# Autodesk Inventor assembly: First Design
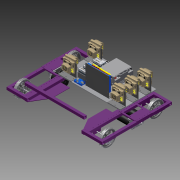
[picture p0: Inventor's stored thumbnail of the model, 180x180]
Saved by Autodesk Inventor 2012 (Build 160160000, 160)
## iProperties
Created: 2012-01-09
Part Number: First Design
Document SubType Name: Assembly
Designer: William
Author: William
## Documents named in this file (12)
- C:\Users\William\Dropbox\Robotics\CAD\team1885frc\Robot2012\Concepts\Electronics Board\First Design.iam
- C:\Users\William\Dropbox\Robotics\CAD\team1885frc\Robot2012\DriveTrain\DiveTrain_FullAssembly.iam
- C:\Users\William\Dropbox\Robotics\CAD\team1885frc\Robot2012\Concepts\Electronics Board\24in-by-14in_electronics_board.ipt
- C:\Users\William\Dropbox\Robotics\CAD\team1885frc\Electronics\Jag\Jag.iam
- C:\Users\William\Dropbox\Robotics\CAD\team1885frc\Electronics\DigitalSidecar\elc_Digital_Sidecar_inv.iam
- C:\Users\William\Dropbox\Robotics\CAD\team1885frc\Electronics\PowerDistributionBoard\elc_Power_Distro_inv.iam
- C:\Users\William\Dropbox\Robotics\CAD\team1885frc\Electronics\Battery.ipt
- C:\Users\William\Dropbox\Robotics\CAD\team1885frc\Robot2012\Concepts\Electronics Board\BatteryMountSide.ipt
- C:\Users\William\Dropbox\Robotics\CAD\team1885frc\Electronics\cRIO_7Slot\NI Controller.iam
- C:\Users\William\Dropbox\Robotics\CAD\team1885frc\Electronics\Breaker\Breaker.iam
- C:\Users\William\Dropbox\Robotics\CAD\team1885frc\Electronics\dualjaguarstand.ipt
- C:\Users\William\Dropbox\Robotics\CAD\team1885frc\Robot2012\Concepts\Electronics Board\PowerDistributionStandmount.ipt
## Components (27 placed, 11 different names)
1. DiveTrain_FullAssembly:1 [sub-assembly] — Flush:2, Angle:1, Angle:9, Flush:27
2. 24in-by-14in_electronics_board:1 — Flush:2, Mate:12, Mate:15, Mate:16, Flush:8, Flush:10, Flush:11, Mate:28, Flush:12, Mate:47, Flush:17, Flush:18, Mate:51, Flush:19, Mate:55, Flush:20, Flush:21, Mate:60, Flush:22, Flush:23, Mate:64, Flush:24, Flush:25, Mate:71, Flush:26, Flush:27
3. Jag:1 [sub-assembly] — Mate:26, Mate:42, Mate:54, Mate:56, Mate:58
4. Jag:2 [sub-assembly] — Mate:27, Mate:41, Mate:53
5. Jag:3 [sub-assembly] — Mate:31, Mate:40, Mate:49, Flush:18
6. Jag:4 [sub-assembly] — Mate:31, Mate:40, Mate:46, Mate:48, Angle:4
7. Jag:5 [sub-assembly] — Mate:35, Mate:39, Mate:65, Mate:66, Mate:67
8. Jag:6 [sub-assembly] — Mate:37, Mate:38, Mate:59, Mate:62, Angle:7
9. Jag:7 [sub-assembly] — Mate:37, Mate:38, Mate:61, Flush:23
10. Jag:8 [sub-assembly] — Mate:27, Mate:41, Mate:50, Mate:52, Mate:58, Angle:5
11. Jag:9 [sub-assembly] — Mate:26, Mate:42, Mate:57, Angle:6
12. Jag:10 [sub-assembly] — Mate:35, Mate:39, Mate:63, Angle:8
13. elc_Digital_Sidecar_inv:1 [sub-assembly] — Mate:15, Flush:10
14. elc_Power_Distro_inv:1 [sub-assembly] — Mate:68, Mate:69, Mate:70
15. Battery:1 — Mate:2, Mate:3, Mate:4, Mate:5, Mate:6, Mate:7, Mate:8, Mate:9, Mate:10, Mate:11, Flush:3, Flush:4
16. BatteryMountSide:1 — Mate:3, Mate:4, Mate:10
17. BatteryMountSide:2 — Mate:6, Mate:9, Mate:11
18. BatteryMountSide:3 — Mate:2, Mate:5, Flush:3
19. BatteryMountSide:4 — Mate:7, Mate:8, Flush:4, Mate:12, Angle:1, Flush:11
20. NI Controller:1 [sub-assembly] — Mate:16, Flush:8
21. Breaker:1 [sub-assembly] — Mate:28, Flush:12
22. dualjaguarstand:1 — Mate:46, Mate:47, Flush:17, Mate:48, Mate:49, Angle:4
23. dualjaguarstand:2 — Mate:50, Mate:51, Mate:52, Mate:53, Flush:19, Angle:5
24. dualjaguarstand:3 — Mate:54, Mate:55, Mate:56, Mate:57, Flush:20, Flush:21, Angle:6
25. dualjaguarstand:4 — Mate:63, Mate:64, Mate:65, Mate:66, Mate:67, Flush:24, Flush:25, Angle:8
26. dualjaguarstand:5 — Mate:59, Mate:60, Flush:22, Mate:61, Mate:62, Angle:7
27. PowerDistributionStandmount:1 — Mate:68, Mate:69, Mate:70, Mate:71, Angle:9, Flush:26
## Relationships (75: Mate 50, Flush 18, Angle 7)
- Flush:2 (-12.7 mm): DiveTrain_FullAssembly:1 ↔ 24in-by-14in_electronics_board:1
- Mate:2 (5.08 mm): Battery:1 ↔ BatteryMountSide:3
- Mate:3 (5.08 mm): Battery:1 ↔ BatteryMountSide:1
- Mate:4: Battery:1 ↔ BatteryMountSide:1
- Mate:5: Battery:1 ↔ BatteryMountSide:3
- Mate:6: Battery:1 ↔ BatteryMountSide:2
- Mate:7: Battery:1 ↔ BatteryMountSide:4
- Mate:8 (5.08 mm): Battery:1 ↔ BatteryMountSide:4
- Mate:9: Battery:1 ↔ BatteryMountSide:2
- Mate:10 (16.51 mm): Battery:1 ↔ BatteryMountSide:1
- Mate:11 (16.51 mm): Battery:1 ↔ BatteryMountSide:2
- Flush:3 (-12.446 mm): Battery:1 ↔ BatteryMountSide:3
- Flush:4 (12.446 mm): Battery:1 ↔ BatteryMountSide:4
- Mate:12: 24in-by-14in_electronics_board:1 ↔ BatteryMountSide:4
- Mate:15: 24in-by-14in_electronics_board:1 ↔ elc_Digital_Sidecar_inv:1
- Mate:16: 24in-by-14in_electronics_board:1 ↔ NI Controller:1
- Flush:8 (12.7 mm): 24in-by-14in_electronics_board:1 ↔ NI Controller:1
- Flush:10 (12.7 mm): 24in-by-14in_electronics_board:1 ↔ elc_Digital_Sidecar_inv:1
- Angle:1 (0 deg): DiveTrain_FullAssembly:1 ↔ BatteryMountSide:4
- Flush:11: 24in-by-14in_electronics_board:1 ↔ BatteryMountSide:4
- Mate:26: Jag:1 ↔ Jag:9
- Mate:27: Jag:2 ↔ Jag:8
- Mate:28: 24in-by-14in_electronics_board:1 ↔ Breaker:1
- Flush:12 (12.7 mm): 24in-by-14in_electronics_board:1 ↔ Breaker:1
- Mate:31: Jag:3 ↔ Jag:4
- Mate:35: Jag:5 ↔ Jag:10
- Mate:37: Jag:6 ↔ Jag:7
- Mate:38: Jag:6 ↔ Jag:7
- Mate:39: Jag:5 ↔ Jag:10
- Mate:40: Jag:3 ↔ Jag:4
- Mate:41: Jag:2 ↔ Jag:8
- Mate:42: Jag:1 ↔ Jag:9
- Mate:46: Jag:4 ↔ dualjaguarstand:1
- Mate:47: 24in-by-14in_electronics_board:1 ↔ dualjaguarstand:1
- Flush:17: 24in-by-14in_electronics_board:1 ↔ dualjaguarstand:1
- Mate:48: Jag:4 ↔ dualjaguarstand:1
- Mate:49: Jag:3 ↔ dualjaguarstand:1
- Angle:4 (0 deg): Jag:4 ↔ dualjaguarstand:1
- Flush:18: 24in-by-14in_electronics_board:1 ↔ Jag:3
- Mate:50: Jag:8 ↔ dualjaguarstand:2
- Mate:51: 24in-by-14in_electronics_board:1 ↔ dualjaguarstand:2
- Mate:52: Jag:8 ↔ dualjaguarstand:2
- Mate:53: Jag:2 ↔ dualjaguarstand:2
- Flush:19: 24in-by-14in_electronics_board:1 ↔ dualjaguarstand:2
- Mate:54: Jag:1 ↔ dualjaguarstand:3
- Mate:55: 24in-by-14in_electronics_board:1 ↔ dualjaguarstand:3
- Mate:56: Jag:1 ↔ dualjaguarstand:3
- Mate:57: Jag:9 ↔ dualjaguarstand:3
- Flush:20: 24in-by-14in_electronics_board:1 ↔ dualjaguarstand:3
- Flush:21: 24in-by-14in_electronics_board:1 ↔ dualjaguarstand:3
- Mate:58 (20.32 mm): Jag:1 ↔ Jag:8
- Mate:59: Jag:6 ↔ dualjaguarstand:5
- Mate:60: 24in-by-14in_electronics_board:1 ↔ dualjaguarstand:5
- Flush:22: 24in-by-14in_electronics_board:1 ↔ dualjaguarstand:5
- Mate:61: Jag:7 ↔ dualjaguarstand:5
- Mate:62: Jag:6 ↔ dualjaguarstand:5
- Angle:5 (0 deg): Jag:8 ↔ dualjaguarstand:2
- Angle:6 (0 deg): Jag:9 ↔ dualjaguarstand:3
- Angle:7 (0 deg): Jag:6 ↔ dualjaguarstand:5
- Flush:23: 24in-by-14in_electronics_board:1 ↔ Jag:7
- Mate:63: Jag:10 ↔ dualjaguarstand:4
- Mate:64: 24in-by-14in_electronics_board:1 ↔ dualjaguarstand:4
- Mate:65: Jag:5 ↔ dualjaguarstand:4
- Mate:66: Jag:5 ↔ dualjaguarstand:4
- Mate:67: Jag:5 ↔ dualjaguarstand:4
- Flush:24: 24in-by-14in_electronics_board:1 ↔ dualjaguarstand:4
- Flush:25: 24in-by-14in_electronics_board:1 ↔ dualjaguarstand:4
- Angle:8 (0 deg): Jag:10 ↔ dualjaguarstand:4
- Mate:68: elc_Power_Distro_inv:1 ↔ PowerDistributionStandmount:1
- Mate:69: elc_Power_Distro_inv:1 ↔ PowerDistributionStandmount:1
- Mate:70: elc_Power_Distro_inv:1 ↔ PowerDistributionStandmount:1
- Mate:71: 24in-by-14in_electronics_board:1 ↔ PowerDistributionStandmount:1
- Angle:9 (0 deg): DiveTrain_FullAssembly:1 ↔ PowerDistributionStandmount:1
- Flush:26 (38.1 mm): 24in-by-14in_electronics_board:1 ↔ PowerDistributionStandmount:1
- Flush:27 (12.7 mm): DiveTrain_FullAssembly:1 ↔ 24in-by-14in_electronics_board:1
